# Autodesk Inventor assembly: swivel_brkt
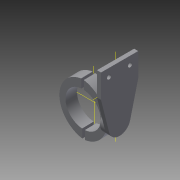
[picture p0: Inventor's stored thumbnail of the model, 180x180]
Saved by Autodesk Inventor 2015 (Build 190159000, 159)
## iProperties
Created: 2015-09-23
Part Number: swivel_brkt
Description: insert description/title
Document SubType Name: Assembly
Designer: francis
Author: francis
Part Category: insert part category and press enter to fill value
## Documents named in this file (3)
- C:\Users\francis\Documents\GitHub\CAD\swivel_brkt.iam
- C:\Users\francis\Documents\GitHub\CAD\collar.ipt
- C:\Users\francis\Documents\GitHub\CAD\turny_bit.ipt
## Components (2 placed, 2 different names)
1. collar:1 — Rotational:1
2. turny_bit:1 — Rotational:1
## Relationships (1: RevoluteJoint 1)
- Rotational:1 [RevoluteJoint] (0.5 mm): collar:1 ↔ turny_bit:1
